# Autodesk Inventor assembly: C-BGHKA6902ZZ-30
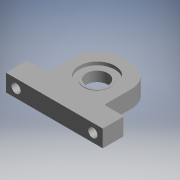
[picture p0: Inventor's stored thumbnail of the model, 180x180]
Saved by Autodesk Inventor 2017.3 (Build 213256000, 256)
## iProperties
Category: PARTsolutions
Company: MISUMI
Part Number: C-BGHKA6902ZZ-30
Catalog Web Link: www.cadenas.de
Description: C-BGHKA-C-VALUE Medium Accuracy Bearings with Housings - T-Shaped
Vendor: MISUMI
Document SubType Name: Assembly
Designer: partserver
Manufacturer: MISUMI
Mass: 22.6591 g
Surface Area: 104.475 cm^2
Volume: 22.6591 cm^3
Density: 1 g/cm^3
Title: C-BGHKA6902ZZ-30
Author: Cadenas PARTsolutions
Comments: C-VALUE Medium Accuracy Bearings with Housings - T-Shaped
PSOL_IDENT_0: {$CADENAS_DATA\23d-libs\misumi\metric\12_bearing_holders\12_cn\c_bghka_asmtab.prj},182 {VTYP=3D},{ST
PSOL_IDENT_1: YP=ASSTAB},{NB=C-BGHKA6902ZZ-30},{LINA=C-BGHKA6902ZZ-30},{NN=C-BGHKA},{DATE=30.06.2021 12:57:54},{GE
PSOL_IDENT_2: OMDATE=06.02.2013},{VERSION=},{LINEID=60},{WBVAR=HH},{WBNUMERIC=HH}  {NB=C-BGHKA6902ZZ-30},{LINA=C-B
PSOL_IDENT_3: GHKA6902ZZ-30},{KT=DUMMY},{PN=C-BGHKA6902ZZ-30},{TYPE=C-BGHKA},{BN=6902ZZ},{HH=30},{HHALG=30,40,50},
PSOL_IDENT_4: {DD=15},{H=50},{L1=54},{DD1=6.5},{L=68},{L2=40},{T=12},{S=15},{DDHH=25},{DH7=28},{B=7},{PPATH=c_bghk
PSOL_IDENT_5: a/c_bghka_asmtpl.prj}
NB: C-BGHKA6902ZZ-30
NN: C-BGHKA
NT: C-VALUE Medium Accuracy Bearings with Housings - T-Shaped
NBSYN: $PN.
LINA: C-BGHKA6902ZZ-30
CATALOG: Misumi
PN: C-BGHKA6902ZZ-30
BN: 6902ZZ
HH: 30
DD: 15
H: 50
L1: 54
DD1: 6.5
L: 68
L2: 40
T: 12
S: 15
DDHH: 25
DH7: 28
B: 7
SUPPLIER: MISUMI
ARTICLENO: C-BGHKA6902ZZ-30
BOMINFO: C-BGHKA6902ZZ-30
CREATOR: CADENAS GmbH
## Documents named in this file (4)
- e:\temp\worker_15\temp\exporttempdir_8812_199_QHdKz\format_0\C-BGHKA6902ZZ-30.iam
- e:\temp\worker_15\temp\exporttempdir_8812_199_QHdKz\format_0\C-BGHKA6902ZZ-30_b_b.ipt
- e:\temp\worker_15\temp\exporttempdir_8812_199_QHdKz\format_0\C6902ZZ.ipt
- e:\temp\worker_15\temp\exporttempdir_8812_199_QHdKz\format_0\RTWN28.ipt
## Components (3 placed, 3 different names)
1. C-BGHKA6902ZZ-30_b_b:1 — to_bearing_XY@1 <-> to_cp1_XY@2, to_bearing_Z@1 <-> to_cp1_Z@2, to_bearing_YZ@1 <-> to_cp1_YZ@2, to_snapring_XY@1 <-> rr_XY@3, to_snapring_Z@1 <-> rr_Z@3, to_snapring_YZ@1 <-> rr_YZ@3
2. C6902ZZ:1 — to_bearing_XY@1 <-> to_cp1_XY@2, to_bearing_Z@1 <-> to_cp1_Z@2, to_bearing_YZ@1 <-> to_cp1_YZ@2
3. RTWN28:1 — to_snapring_XY@1 <-> rr_XY@3, to_snapring_Z@1 <-> rr_Z@3, to_snapring_YZ@1 <-> rr_YZ@3
## Relationships (6: Mate 3, Angle 2, Flush 1)
- to_bearing_XY@1 <-> to_cp1_XY@2 [Flush]: C-BGHKA6902ZZ-30_b_b:1 ↔ C6902ZZ:1
- to_bearing_Z@1 <-> to_cp1_Z@2 [Mate]: C-BGHKA6902ZZ-30_b_b:1 ↔ C6902ZZ:1
- to_bearing_YZ@1 <-> to_cp1_YZ@2 [Angle] (0 deg): C-BGHKA6902ZZ-30_b_b:1 ↔ C6902ZZ:1
- to_snapring_XY@1 <-> rr_XY@3 [Mate]: C-BGHKA6902ZZ-30_b_b:1 ↔ RTWN28:1
- to_snapring_Z@1 <-> rr_Z@3 [Mate]: C-BGHKA6902ZZ-30_b_b:1 ↔ RTWN28:1
- to_snapring_YZ@1 <-> rr_YZ@3 [Angle] (0 deg): C-BGHKA6902ZZ-30_b_b:1 ↔ RTWN28:1
